# Autodesk Inventor assembly: dashboard_assembly
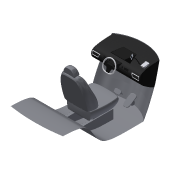
[picture p0: Inventor's stored thumbnail of the model, 180x180]
Saved by Autodesk Inventor 2019 (Build 230136000, 136)
## iProperties
Created: 2018-11-23
Part Number: dashboard_assembly
Material: Generic
Document SubType Name: Assembly
Designer: cadcae
Author: cadcae
## Documents named in this file (3)
- C:\Users\CADCAE\Downloads\3D_real\dashboard_assembly.iam
- C:\Users\CADCAE\Downloads\3D_real\Auto\UNO interior concept.ipt
- C:\Users\CADCAE\Downloads\3D_real\modelo_completo.iam
## Components (2 placed, 2 different names)
1. UNO interior concept:1 — Flush:1, Flush:2, Flush:3, Mate:1, Angle:3
2. modelo_completo:1 [sub-assembly] — Angle:1, Mate:2
## Relationships (8: Flush 4, Angle 2, Mate 2)
- Flush:1: UNO interior concept:1
- Flush:2: UNO interior concept:1
- Flush:3: UNO interior concept:1
- Angle:1 (0 deg): modelo_completo:1
- Mate:1: UNO interior concept:1
- Angle:3 (170 deg): UNO interior concept:1
- Flush:4 (34.25 mm)
- Mate:2: modelo_completo:1
